# Autodesk Inventor assembly: version3
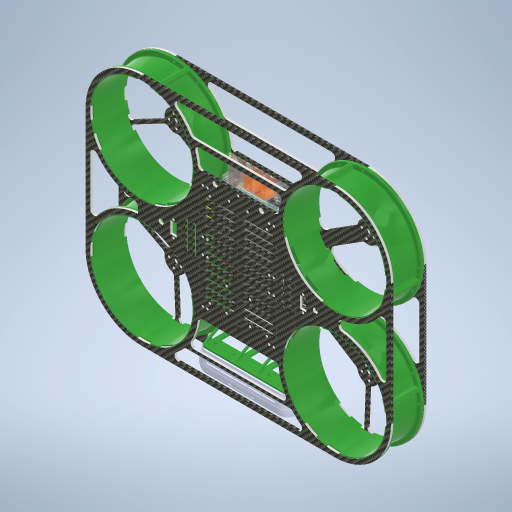
[picture p0: Inventor's stored thumbnail of the model, 512x512]
Saved by Autodesk Inventor 2024 (Build 280153000, 153)
## iProperties
Created: 2025-03-08
Part Number: version3
Document SubType Name: Assembly
Designer: Bruno
Author: Bruno
## Documents named in this file (9)
- D:\Work\Research\Repositories\CybAer\pegasus_cad\models\version3\version3.iam
- D:\Work\Research\Repositories\CybAer\pegasus_cad\models\version3\v3_top_carbon_fiber.ipt
- D:\Work\Research\Repositories\CybAer\pegasus_cad\models\version3\OrinNanoSDK-P3767ENVELOPE_noBase.ipt
- D:\Work\Research\Repositories\CybAer\pegasus_cad\models\version3\spacer-5mm_2-6.ipt
- D:\Work\Research\Repositories\CybAer\pegasus_cad\models\version3\v3_bottom_carbon_fiber.ipt
- D:\Work\Research\Repositories\CybAer\pegasus_cad\models\version3\v3_prop_guard.ipt
- D:\Work\Research\Repositories\CybAer\pegasus_cad\models\version3\v3_realsense_mount.ipt
- D:\Work\Research\Repositories\CybAer\pegasus_cad\models\version3\D455_Solid.ipt
- D:\Work\Research\Repositories\CybAer\pegasus_cad\models\version3\XT60E-M.ipt
## Components (14 placed, 8 different names)
1. v3_bottom_carbon_fiber:1 — Insert:11, Insert:12, Mate:9, Insert:16, Mate:15, Insert:20, Insert:21, Insert:25, Insert:27, Mate:16
2. OrinNanoSDK-P3767ENVELOPE_noBase:1 — Insert:1, Insert:2, Insert:3
3. spacer-5mm_2-6:1 — Insert:2, Mate:15
4. spacer-5mm_2-6:2 — Insert:1
5. spacer-5mm_2-6:3
6. spacer-5mm_2-6:4 — Insert:3
7. v3_top_carbon_fiber:1 — Insert:18, Insert:26
8. v3_prop_guard:1 — Insert:11, Insert:18
9. v3_prop_guard:2 — Insert:16, Insert:26
10. v3_prop_guard:3 — Insert:12, Mate:9
11. v3_prop_guard:4 — Insert:25
12. v3_realsense_mount:1 — Insert:20, Insert:21, Insert:22, Insert:23
13. D455_Solid:1 — Insert:22, Insert:23
14. XT60E-M:1 — Insert:27, Mate:16
## Relationships (23: Insert 15, Mate 7, Flush 1)
- [Flush]: v3_bottom_carbon_fiber:1
- [Mate]: v3_bottom_carbon_fiber:1
- [Mate]: v3_bottom_carbon_fiber:1
- Insert:1: OrinNanoSDK-P3767ENVELOPE_noBase:1 ↔ spacer-5mm_2-6:2
- Insert:2: OrinNanoSDK-P3767ENVELOPE_noBase:1 ↔ spacer-5mm_2-6:1
- Insert:3: OrinNanoSDK-P3767ENVELOPE_noBase:1 ↔ spacer-5mm_2-6:4
- [Mate]: v3_bottom_carbon_fiber:1 ↔ spacer-5mm_2-6:1
- [Insert]: v3_bottom_carbon_fiber:1 ↔ spacer-5mm_2-6:3
- [Mate]: v3_bottom_carbon_fiber:1 ↔ spacer-5mm_2-6:4
- Insert:11: v3_bottom_carbon_fiber:1 ↔ v3_prop_guard:1
- Insert:12: v3_bottom_carbon_fiber:1 ↔ v3_prop_guard:3
- Mate:9: v3_bottom_carbon_fiber:1 ↔ v3_prop_guard:3
- Insert:16: v3_bottom_carbon_fiber:1 ↔ v3_prop_guard:2
- Insert:18: v3_top_carbon_fiber:1 ↔ v3_prop_guard:1
- Mate:15: v3_bottom_carbon_fiber:1 ↔ spacer-5mm_2-6:1
- Insert:20: v3_bottom_carbon_fiber:1 ↔ v3_realsense_mount:1
- Insert:21: v3_bottom_carbon_fiber:1 ↔ v3_realsense_mount:1
- Insert:22: v3_realsense_mount:1 ↔ D455_Solid:1
- Insert:23: v3_realsense_mount:1 ↔ D455_Solid:1
- Insert:25: v3_bottom_carbon_fiber:1 ↔ v3_prop_guard:4
- Insert:26: v3_top_carbon_fiber:1 ↔ v3_prop_guard:2
- Insert:27: v3_bottom_carbon_fiber:1 ↔ XT60E-M:1
- Mate:16: v3_bottom_carbon_fiber:1 ↔ XT60E-M:1
